# Autodesk Inventor assembly: sparAssembly
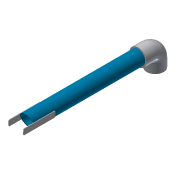
[picture p0: Inventor's stored thumbnail of the model, 180x180]
Saved by Autodesk Inventor 2016 (Build 200138000, 138)
## iProperties
Created: 2013-12-03
Part Number: sparAssembly
Document SubType Name: Assembly
Designer: Dave
Author: Dave
## Documents named in this file (5)
- C:\Users\krosie\Google Drive\HERA\hera-cad\support\sparAssembly.iam
- C:\Users\krosie\Google Drive\HERA\hera-cad\surface\joinerBracket.ipt
- C:\Users\krosie\Google Drive\HERA\hera-cad\smallParts\elbow_90deg_63mm.ipt
- C:\Users\krosie\Google Drive\HERA\hera-cad\support\sparVert_C.ipt
- sparVert_C.ipt
## Components (4 placed, 3 different names)
1. sparVert_C:1 — Insert:1, Insert:2, Insert:3
2. elbow_90deg_63mm:1 — Insert:1
3. joinerBracket:1 — Insert:2, Insert:3
4. joinerBracket:2
## Component patterns: (2 elements, first: joinerBracket:1)
## Relationships (3: Insert 3)
- Insert:1 (-38 mm): sparVert_C:1 ↔ elbow_90deg_63mm:1
- Insert:2: sparVert_C:1 ↔ joinerBracket:1
- Insert:3: sparVert_C:1 ↔ joinerBracket:1
